# Autodesk Inventor assembly: chain(a)
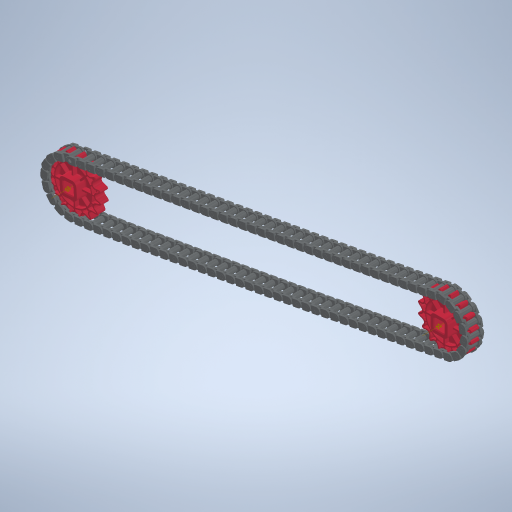
[picture p0: Inventor's stored thumbnail of the model, 512x512]
Saved by Autodesk Inventor 2023 (Build 270158000, 158)
## iProperties
Created: 2022-08-08
Part Number: chain(a)
Document SubType Name: Assembly
Designer: aaron
Author: aaron
## Documents named in this file (3)
- C:\Users\aaron\Documents\Inventor\Spin Up\library\Motion\New Sprockets\chain(aB).iam
- C:\Users\aaron\Documents\Inventor\Spin Up\library\Motion\New Sprockets\16T.ipt
- C:\Users\aaron\Documents\Inventor\Spin Up\library\Motion\New Sprockets\IQ chain.ipt
## Components (96 placed, 2 different names)
1. 16T:1 — Mate:1, Flush:1, Flush:2, Mate:65, Mate:86, Mate:87, Mate:88, Mate:89, Mate:90, Mate:91, Mate:92, Mate:93, Mate:112
2. 16T:2 — Mate:1, Flush:1, Flush:2, Mate:67, Mate:68, Mate:81, Mate:82, Mate:83, Mate:84, Mate:85, Mate:111, Flush:94
3. IQ chain:1 — Mate:2, Flush:3, Mate:64, Flush:65
4. IQ chain:2 — Mate:2, Flush:3, Mate:4, Flush:5
5. IQ chain:3 — Mate:4, Flush:5, Mate:114, Flush:95
6. IQ chain:5 — Mate:114, Flush:95
7. IQ chain:6
8. IQ chain:7
9. IQ chain:8 — Mate:16, Flush:17
10. IQ chain:9 — Mate:16, Flush:17
11. IQ chain:10
12. IQ chain:11
13. IQ chain:12
14. IQ chain:13
15. IQ chain:14
16. IQ chain:15
17. IQ chain:16 — Mate:32, Flush:33
18. IQ chain:17 — Mate:32, Flush:33
19. IQ chain:18
20. IQ chain:19
21. IQ chain:20
22. IQ chain:21
23. IQ chain:22
24. IQ chain:23
25. IQ chain:24
26. IQ chain:25 — Mate:113
27. IQ chain:27 — Mate:113
28. IQ chain:28
29. IQ chain:29 — Mate:120, Flush:99
30. IQ chain:30
31. IQ chain:31 — Mate:67
32. IQ chain:32 — Mate:68, Mate:80, Flush:77
33. IQ chain:33 — Mate:100, Flush:84
34. IQ chain:34
35. IQ chain:35 — Mate:116
36. IQ chain:37 — Mate:117
37. IQ chain:38
38. IQ chain:39
39. IQ chain:40
40. IQ chain:41
41. IQ chain:42
42. IQ chain:43
43. IQ chain:44
44. IQ chain:45
45. IQ chain:46
46. IQ chain:47
47. IQ chain:48 — Mate:93
48. IQ chain:49 — Mate:92
49. IQ chain:50 — Mate:91
50. IQ chain:51 — Mate:90
51. IQ chain:52 — Mate:89
52. IQ chain:53 — Mate:88
53. IQ chain:54 — Mate:87
54. IQ chain:55 — Mate:86
55. IQ chain:56 — Mate:65
56. IQ chain:57 — Mate:112
57. IQ chain:58
58. IQ chain:59
59. IQ chain:60
60. IQ chain:61
61. IQ chain:62
62. IQ chain:63
63. IQ chain:64 — Mate:64, Flush:65
64. IQ chain:65 — Mate:80, Flush:77, Mate:81
65. IQ chain:66 — Mate:82
66. IQ chain:67 — Mate:83
67. IQ chain:68 — Mate:84
68. IQ chain:69 — Mate:85, Flush:94
69. IQ chain:70 — Mate:111
70. IQ chain:71
71. IQ chain:72
72. IQ chain:73
73. IQ chain:74
74. IQ chain:75
75. IQ chain:76 — Mate:109, Flush:93
76. IQ chain:77 — Mate:108, Flush:92
77. IQ chain:78
78. IQ chain:79
79. IQ chain:80
80. IQ chain:81
81. IQ chain:82
82. IQ chain:83 — Mate:100, Flush:84
83. IQ chain:84 — Mate:108, Flush:92
84. IQ chain:85 — Mate:110
85. IQ chain:86
86. IQ chain:87
87. IQ chain:88
88. IQ chain:89
89. IQ chain:90
90. IQ chain:91
91. IQ chain:92 — Mate:109, Flush:93, Mate:110
92. IQ chain:93 — Mate:116
93. IQ chain:94 — Mate:117
94. IQ chain:95 — Mate:120, Flush:99
95. IQ chain:96 — Flush:100
96. IQ chain:97 — Flush:100
## Relationships (206: Mate 112, Flush 94)
- Mate:1 (248.793 mm): 16T:1 ↔ 16T:2
- Flush:1: 16T:1 ↔ 16T:2
- Flush:2: 16T:1 ↔ 16T:2
- Mate:2: IQ chain:1 ↔ IQ chain:2
- Flush:3: IQ chain:1 ↔ IQ chain:2
- Mate:4: IQ chain:2 ↔ IQ chain:3
- Flush:5: IQ chain:2 ↔ IQ chain:3
- [Mate]: IQ chain:5 ↔ IQ chain:6
- [Flush]: IQ chain:5 ↔ IQ chain:6
- [Mate]: IQ chain:7 ↔ IQ chain:8
- [Flush]: IQ chain:7 ↔ IQ chain:8
- [Mate]: IQ chain:6 ↔ IQ chain:7
- [Flush]: IQ chain:6 ↔ IQ chain:7
- [Mate]: IQ chain:9 ↔ IQ chain:10
- [Flush]: IQ chain:9 ↔ IQ chain:10
- [Mate]: IQ chain:11 ↔ IQ chain:12
- [Flush]: IQ chain:11 ↔ IQ chain:12
- [Mate]: IQ chain:10 ↔ IQ chain:11
- [Flush]: IQ chain:10 ↔ IQ chain:11
- [Mate]: IQ chain:13 ↔ IQ chain:14
- [Flush]: IQ chain:13 ↔ IQ chain:14
- [Mate]: IQ chain:15 ↔ IQ chain:16
- [Flush]: IQ chain:15 ↔ IQ chain:16
- [Mate]: IQ chain:14 ↔ IQ chain:15
- [Flush]: IQ chain:14 ↔ IQ chain:15
- [Mate]: IQ chain:12 ↔ IQ chain:13
- [Flush]: IQ chain:12 ↔ IQ chain:13
- Mate:16: IQ chain:8 ↔ IQ chain:9
- Flush:17: IQ chain:8 ↔ IQ chain:9
- [Mate]: IQ chain:17 ↔ IQ chain:18
- [Flush]: IQ chain:17 ↔ IQ chain:18
- [Mate]: IQ chain:19 ↔ IQ chain:20
- [Flush]: IQ chain:19 ↔ IQ chain:20
- [Mate]: IQ chain:18 ↔ IQ chain:19
- [Flush]: IQ chain:18 ↔ IQ chain:19
- [Mate]: IQ chain:21 ↔ IQ chain:22
- [Flush]: IQ chain:21 ↔ IQ chain:22
- [Mate]: IQ chain:23 ↔ IQ chain:24
- [Flush]: IQ chain:23 ↔ IQ chain:24
- [Mate]: IQ chain:22 ↔ IQ chain:23
- [Flush]: IQ chain:22 ↔ IQ chain:23
- [Mate]: IQ chain:20 ↔ IQ chain:21
- [Flush]: IQ chain:20 ↔ IQ chain:21
- [Mate]: IQ chain:27 ↔ IQ chain:28
- [Flush]: IQ chain:27 ↔ IQ chain:28
- [Flush]: IQ chain:29 ↔ IQ chain:30
- [Mate]: IQ chain:31 ↔ IQ chain:32
- [Flush]: IQ chain:31 ↔ IQ chain:32
- [Mate]: IQ chain:30 ↔ IQ chain:31
- [Flush]: IQ chain:30 ↔ IQ chain:31
- [Mate]: IQ chain:28 ↔ IQ chain:29
- [Flush]: IQ chain:28 ↔ IQ chain:29
- [Mate]: IQ chain:24 ↔ IQ chain:25
- [Flush]: IQ chain:24 ↔ IQ chain:25
- Mate:32: IQ chain:16 ↔ IQ chain:17
- Flush:33: IQ chain:16 ↔ IQ chain:17
- [Mate]: IQ chain:33 ↔ IQ chain:34
- [Flush]: IQ chain:33 ↔ IQ chain:34
- [Mate]: IQ chain:34 ↔ IQ chain:35
- [Flush]: IQ chain:34 ↔ IQ chain:35
- [Mate]: IQ chain:37 ↔ IQ chain:38
- [Flush]: IQ chain:37 ↔ IQ chain:38
- [Mate]: IQ chain:39 ↔ IQ chain:40
- [Flush]: IQ chain:39 ↔ IQ chain:40
- [Mate]: IQ chain:38 ↔ IQ chain:39
- [Flush]: IQ chain:38 ↔ IQ chain:39
- [Mate]: IQ chain:41 ↔ IQ chain:42
- [Flush]: IQ chain:41 ↔ IQ chain:42
- [Mate]: IQ chain:43 ↔ IQ chain:44
- [Flush]: IQ chain:43 ↔ IQ chain:44
- [Mate]: IQ chain:42 ↔ IQ chain:43
- [Flush]: IQ chain:42 ↔ IQ chain:43
- [Mate]: IQ chain:45 ↔ IQ chain:46
- [Flush]: IQ chain:45 ↔ IQ chain:46
- [Mate]: IQ chain:47 ↔ IQ chain:48
- [Flush]: IQ chain:47 ↔ IQ chain:48
- [Mate]: IQ chain:46 ↔ IQ chain:47
- [Flush]: IQ chain:46 ↔ IQ chain:47
- [Mate]: IQ chain:44 ↔ IQ chain:45
- [Flush]: IQ chain:44 ↔ IQ chain:45
- [Mate]: IQ chain:40 ↔ IQ chain:41
- [Flush]: IQ chain:40 ↔ IQ chain:41
- [Mate]: IQ chain:49 ↔ IQ chain:50
- [Flush]: IQ chain:49 ↔ IQ chain:50
- [Mate]: IQ chain:51 ↔ IQ chain:52
- [Flush]: IQ chain:51 ↔ IQ chain:52
- [Mate]: IQ chain:50 ↔ IQ chain:51
- [Flush]: IQ chain:50 ↔ IQ chain:51
- [Mate]: IQ chain:53 ↔ IQ chain:54
- [Flush]: IQ chain:53 ↔ IQ chain:54
- [Mate]: IQ chain:55 ↔ IQ chain:56
- [Flush]: IQ chain:55 ↔ IQ chain:56
- [Mate]: IQ chain:54 ↔ IQ chain:55
- [Flush]: IQ chain:54 ↔ IQ chain:55
- [Mate]: IQ chain:52 ↔ IQ chain:53
- [Flush]: IQ chain:52 ↔ IQ chain:53
- [Mate]: IQ chain:57 ↔ IQ chain:58
- [Flush]: IQ chain:57 ↔ IQ chain:58
- [Mate]: IQ chain:59 ↔ IQ chain:60
- [Flush]: IQ chain:59 ↔ IQ chain:60
- [Mate]: IQ chain:58 ↔ IQ chain:59
- [Flush]: IQ chain:58 ↔ IQ chain:59
- [Mate]: IQ chain:61 ↔ IQ chain:62
- [Flush]: IQ chain:61 ↔ IQ chain:62
- [Mate]: IQ chain:63 ↔ IQ chain:64
- [Flush]: IQ chain:63 ↔ IQ chain:64
- [Mate]: IQ chain:62 ↔ IQ chain:63
- [Flush]: IQ chain:62 ↔ IQ chain:63
- [Mate]: IQ chain:60 ↔ IQ chain:61
- [Flush]: IQ chain:60 ↔ IQ chain:61
- [Mate]: IQ chain:56 ↔ IQ chain:57
- [Flush]: IQ chain:56 ↔ IQ chain:57
- [Mate]: IQ chain:48 ↔ IQ chain:49
- [Flush]: IQ chain:48 ↔ IQ chain:49
- Mate:64: IQ chain:1 ↔ IQ chain:64
- Flush:65: IQ chain:1 ↔ IQ chain:64
- Mate:65: 16T:1 ↔ IQ chain:56
- Mate:67: 16T:2 ↔ IQ chain:31
- Mate:68: 16T:2 ↔ IQ chain:32
- [Mate]: IQ chain:66 ↔ IQ chain:67
- [Flush]: IQ chain:66 ↔ IQ chain:67
- [Mate]: IQ chain:68 ↔ IQ chain:69
- [Flush]: IQ chain:68 ↔ IQ chain:69
- [Mate]: IQ chain:67 ↔ IQ chain:68
- [Flush]: IQ chain:67 ↔ IQ chain:68
- [Mate]: IQ chain:70 ↔ IQ chain:71
- [Flush]: IQ chain:70 ↔ IQ chain:71
- [Mate]: IQ chain:72 ↔ IQ chain:73
- [Flush]: IQ chain:72 ↔ IQ chain:73
- [Mate]: IQ chain:71 ↔ IQ chain:72
- [Flush]: IQ chain:71 ↔ IQ chain:72
- [Mate]: IQ chain:69 ↔ IQ chain:70
- [Flush]: IQ chain:69 ↔ IQ chain:70
- [Mate]: IQ chain:65 ↔ IQ chain:66
- [Flush]: IQ chain:65 ↔ IQ chain:66
- [Mate]: IQ chain:74 ↔ IQ chain:75
- [Flush]: IQ chain:74 ↔ IQ chain:75
- [Mate]: IQ chain:75 ↔ IQ chain:76
- [Flush]: IQ chain:75 ↔ IQ chain:76
- [Mate]: IQ chain:73 ↔ IQ chain:74
- [Flush]: IQ chain:73 ↔ IQ chain:74
- Mate:80: IQ chain:32 ↔ IQ chain:65
- Flush:77: IQ chain:32 ↔ IQ chain:65
- Mate:81: 16T:2 ↔ IQ chain:65
- Mate:82: 16T:2 ↔ IQ chain:66
- Mate:83: 16T:2 ↔ IQ chain:67
- Mate:84: 16T:2 ↔ IQ chain:68
- Mate:85: 16T:2 ↔ IQ chain:69
- Mate:86: 16T:1 ↔ IQ chain:55
- Mate:87: 16T:1 ↔ IQ chain:54
- Mate:88: 16T:1 ↔ IQ chain:53
- Mate:89: 16T:1 ↔ IQ chain:52
- Mate:90: 16T:1 ↔ IQ chain:51
- Mate:91: 16T:1 ↔ IQ chain:50
- Mate:92: 16T:1 ↔ IQ chain:49
- Mate:93: 16T:1 ↔ IQ chain:48
- [Mate]: IQ chain:77 ↔ IQ chain:78
- [Flush]: IQ chain:77 ↔ IQ chain:78
- [Mate]: IQ chain:79 ↔ IQ chain:80
- [Flush]: IQ chain:79 ↔ IQ chain:80
- [Mate]: IQ chain:78 ↔ IQ chain:79
- [Flush]: IQ chain:78 ↔ IQ chain:79
- [Mate]: IQ chain:81 ↔ IQ chain:82
- [Flush]: IQ chain:81 ↔ IQ chain:82
- [Mate]: IQ chain:82 ↔ IQ chain:83
- [Flush]: IQ chain:82 ↔ IQ chain:83
- [Mate]: IQ chain:80 ↔ IQ chain:81
- [Flush]: IQ chain:80 ↔ IQ chain:81
- Mate:100: IQ chain:33 ↔ IQ chain:83
- Flush:84: IQ chain:33 ↔ IQ chain:83
- [Mate]: IQ chain:85 ↔ IQ chain:86
- [Flush]: IQ chain:85 ↔ IQ chain:86
- [Mate]: IQ chain:87 ↔ IQ chain:88
- [Flush]: IQ chain:87 ↔ IQ chain:88
- [Mate]: IQ chain:86 ↔ IQ chain:87
- [Flush]: IQ chain:86 ↔ IQ chain:87
- [Mate]: IQ chain:89 ↔ IQ chain:90
- [Flush]: IQ chain:89 ↔ IQ chain:90
- [Mate]: IQ chain:90 ↔ IQ chain:91
- [Flush]: IQ chain:90 ↔ IQ chain:91
- [Mate]: IQ chain:88 ↔ IQ chain:89
- [Flush]: IQ chain:88 ↔ IQ chain:89
- [Mate]: IQ chain:84 ↔ IQ chain:91
- [Flush]: IQ chain:84 ↔ IQ chain:91
- Mate:108: IQ chain:77 ↔ IQ chain:84
- Flush:92: IQ chain:77 ↔ IQ chain:84
- Mate:109: IQ chain:76 ↔ IQ chain:92
- Flush:93: IQ chain:76 ↔ IQ chain:92
- Mate:110: IQ chain:85 ↔ IQ chain:92
- Mate:111: 16T:2 ↔ IQ chain:70
- Flush:94: 16T:2 ↔ IQ chain:69
- Mate:112: 16T:1 ↔ IQ chain:57
- Mate:113: IQ chain:25 ↔ IQ chain:27
- Mate:114: IQ chain:3 ↔ IQ chain:5
- Flush:95: IQ chain:3 ↔ IQ chain:5
- [Mate]: IQ chain:93 ↔ IQ chain:94
- [Flush]: IQ chain:93 ↔ IQ chain:94
- Mate:116: IQ chain:35 ↔ IQ chain:93
- Mate:117: IQ chain:37 ↔ IQ chain:94
- [Mate]: IQ chain:95 ↔ IQ chain:96
- [Flush]: IQ chain:95 ↔ IQ chain:96
- [Mate]: IQ chain:96 ↔ IQ chain:97
- [Flush]: IQ chain:96 ↔ IQ chain:97
- Mate:120: IQ chain:29 ↔ IQ chain:95
- Flush:99: IQ chain:29 ↔ IQ chain:95
- Flush:100: IQ chain:96 ↔ IQ chain:97
## Named parameters: d9_d3 = 0 mm, d10_d4 = 0 mm, d11_d5_d3 = 0 mm, d12_d6_d4 = 0 mm, d13_d7 = 0 mm, d14_d8 = 0 mm, d17_d3 = 0 mm, d18_d4 = 0 mm, d19_d5_d3 = 0 mm, d20_d6_d4 = 0 mm, d21_d7 = 0 mm, d22_d8 = 0 mm, d23_d9_d3 = 0 mm, d24_d10_d4 = 0 mm, d25_d11_d5_d3 = 0 mm, d26_d12_d6_d4 = 0 mm, d27_d13_d7 = 0 mm, d28_d14_d8 = 0 mm, d29_d15 = 0 mm, d30_d16 = 0 mm, d33_d32 = 0 mm, d34_d3 = 0 mm, d35_d4 = 0 mm, d36_d5_d3 = 0 mm, d37_d6_d4 = 0 mm, d38_d7 = 0 mm, d39_d8 = 0 mm, d40_d9_d3 = 0 mm, d41_d10_d4 = 0 mm, d42_d11_d5_d3 = 0 mm, d43_d12_d6_d4 = 0 mm, d44_d13_d7 = 0 mm, d45_d14_d8 = 0 mm, d46_d15 = 0 mm, d47_d16 = 0 mm, d50_d19_d5_d3 = 0 mm, d51_d20_d6_d4 = 0 mm, d55_d24_d10_d4 = 0 mm, d56_d25_d11_d5_d3 = 0 mm, d57_d26_d12_d6_d4 = 0 mm, d58_d27_d13_d7 = 0 mm, d59_d28_d14_d8 = 0 mm, d60_d29_d15 = 0 mm, d61_d30_d16 = 0 mm, d62_d31 = 0 mm, d65_d32 = 0 mm, d66_d33_d32 = 0 mm, d67_d34_d3 = 0 mm, d68_d35_d4 = 0 mm, d69_d36_d5_d3 = 0 mm, d70_d37_d6_d4 = 0 mm, d71_d38_d7 = 0 mm, d72_d39_d8 = 0 mm, d73_d40_d9_d3 = 0 mm, d74_d41_d10_d4 = 0 mm, d75_d42_d11_d5_d3 = 0 mm, d76_d43_d12_d6_d4 = 0 mm, d77_d44_d13_d7 = 0 mm, d78_d45_d14_d8 = 0 mm, d79_d46_d15 = 0 mm, d80_d47_d16 = 0 mm, d81_d48_d17_d3 = 0 mm, d82_d49_d18_d4 = 0 mm, d83_d50_d19_d5_d3 = 0 mm, d84_d51_d20_d6_d4 = 0 mm, d85_d52_d21_d7 = 0 mm, d86_d53_d22_d8 = 0 mm, d87_d54_d23_d9_d3 = 0 mm, d88_d55_d24_d10_d4 = 0 mm, d89_d56_d25_d11_d5_d3 = 0 mm, d90_d57_d26_d12_d6_d4 = 0 mm, d91_d58_d27_d13_d7 = 0 mm, d92_d59_d28_d14_d8 = 0 mm, d93_d60_d29_d15 = 0 mm, d94_d61_d30_d16 = 0 mm, d95_d62_d31 = 0 mm, d96_d63 = 0 mm, d97_d64 = 0 mm, d98_d3 = 0 mm, d99_d4 = 0 mm, d102_d7 = 0 mm, d103_d8 = 0 mm, d104_d9_d3 = 0 mm, d105_d10_d4 = 0 mm, d106_d11_d5_d3 = 0 mm, d107_d12_d6_d4 = 0 mm, d108_d13_d7 = 0 mm, d109_d14_d8 = 0 mm, d112_d17_d3 = 0 mm, d113_d18_d4 = 0 mm, d114_d19_d5_d3 = 0 mm, d115_d20_d6_d4 = 0 mm, d116_d21_d7 = 0 mm, d117_d22_d8 = 0 mm, d118_d23_d9_d3 = 0 mm, d119_d24_d10_d4 = 0 mm, d120_d25_d11_d5_d3 = 0 mm, d121_d26_d12_d6_d4 = 0 mm, d122_d27_d13_d7 = 0 mm, d123_d28_d14_d8 = 0 mm, d124_d29_d15 = 0 mm, d125_d30_d16 = 0 mm, d126_d31 = 0 mm, d133_d32 = 0 mm, d134_d34_d3 = 0 mm, d135_d35_d4 = 0 mm, d136_d38_d7 = 0 mm, d137_d39_d8 = 0 mm, d138_d63 = 0 mm, d139_d64 = 0 mm, d140_d17_d3 = 0 mm, d141_d18_d4 = 0 mm, d142_d19_d5_d3 = 0 mm, d143_d20_d6_d4 = 0 mm, d144_d21_d7 = 0 mm, d145_d22_d8 = 0 mm, d146_d23_d9_d3 = 0 mm, d147_d24_d10_d4 = 0 mm, d148_d25_d11_d5_d3 = 0 mm, d149_d26_d12_d6_d4 = 0 mm, d150_d27_d13_d7 = 0 mm, d151_d28_d14_d8 = 0 mm, d152_d29_d15 = 0 mm, d153_d30_d16 = 0 mm, d154_d31 = 0 mm, d170_d98_d3 = 0 mm, d171_d99_d4 = 0 mm, d172_d100_d5_d3 = 0 mm, d173_d101_d6_d4 = 0 mm, d174_d102_d7 = 0 mm, d175_d103_d8 = 0 mm, d176_d104_d9_d3 = 0 mm, d177_d105_d10_d4 = 0 mm, d178_d108_d13_d7 = 0 mm, d179_d109_d14_d8 = 0 mm, d180_d110_d15 = 0 mm, d181_d111_d16 = 0 mm, d184_d170_d98_d3 = 0 mm, d185_d171_d99_d4 = 0 mm, d186_d172_d100_d5_d3 = 0 mm, d187_d173_d101_d6_d4 = 0 mm, d188_d174_d102_d7 = 0 mm, d189_d175_d103_d8 = 0 mm, d190_d176_d104_d9_d3 = 0 mm, d191_d177_d105_d10_d4 = 0 mm, d192_d178_d108_d13_d7 = 0 mm, d193_d179_d109_d14_d8 = 0 mm, d194_d180_d110_d15 = 0 mm, d195_d181_d111_d16 = 0 mm, d196_d182 = 0 mm, d197_d183 = 0 mm, d209_d102_d7 = 0 mm, d210_d103_d8 = 0 mm, d213_d50_d19_d5_d3 = 0 mm, d214_d51_d20_d6_d4 = 0 mm, d215_d60_d29_d15 = 0 mm, d216_d61_d30_d16 = 0 mm
